# Autodesk Inventor assembly: ring_assembly
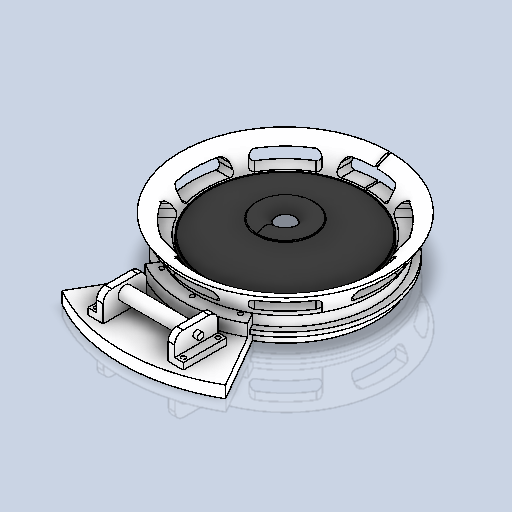
[picture p0: Inventor's stored thumbnail of the model, 512x512]
Saved by Autodesk Inventor 2026.1 (Build 301233000, 233)
## iProperties
Created: 2025-08-31
Part Number: ring_assembly
Document SubType Name: Assembly
Designer: baseb
Author: baseb
## Documents named in this file (7)
- C:\Users\baseb\Desktop\LANL-Glovebox-Closure-Mechanism\ring_assembly.iam
- C:\Users\baseb\Desktop\LANL-Glovebox-Closure-Mechanism\Glove_ring.ipt
- C:\Users\baseb\Desktop\LANL-Glovebox-Closure-Mechanism\shelf_attachment.ipt
- C:\Users\baseb\Desktop\LANL-Glovebox-Closure-Mechanism\drum_holder.ipt
- C:\Users\baseb\Desktop\LANL-Glovebox-Closure-Mechanism\drum.ipt
- C:\Users\baseb\Desktop\LANL-Glovebox-Closure-Mechanism\rubber_sleeve.ipt
- C:\Users\baseb\Desktop\LANL-Glovebox-Closure-Mechanism\rubber_sleeve_open.ipt
## Components (7 placed, 6 different names)
1. Glove_ring:1 — Mate:1, Flush:1, Mate:10, Mate:11, Mate:12, Mate:13
2. shelf_attachment:1 — Mate:1, Flush:1, Mate:2, Mate:3, Mate:4, Mate:5, Mate:6, Mate:7
3. drum_holder:1 — Mate:5, Mate:6, Mate:7
4. drum_holder:2 — Mate:2, Mate:3, Mate:4, Mate:8, Mate:9
5. drum:1 — Mate:8, Mate:9
6. rubber_sleeve:1 — Mate:10, Mate:11
7. rubber_sleeve_open:1 — Mate:12, Mate:13
## Relationships (14: Mate 13, Flush 1)
- Mate:1: Glove_ring:1 ↔ shelf_attachment:1
- Flush:1: Glove_ring:1 ↔ shelf_attachment:1
- Mate:2: shelf_attachment:1 ↔ drum_holder:2
- Mate:3: shelf_attachment:1 ↔ drum_holder:2
- Mate:4: shelf_attachment:1 ↔ drum_holder:2
- Mate:5: shelf_attachment:1 ↔ drum_holder:1
- Mate:6: shelf_attachment:1 ↔ drum_holder:1
- Mate:7: shelf_attachment:1 ↔ drum_holder:1
- Mate:8: drum_holder:2 ↔ drum:1
- Mate:9: drum_holder:2 ↔ drum:1
- Mate:10: Glove_ring:1 ↔ rubber_sleeve:1
- Mate:11: Glove_ring:1 ↔ rubber_sleeve:1
- Mate:12: Glove_ring:1 ↔ rubber_sleeve_open:1
- Mate:13: Glove_ring:1 ↔ rubber_sleeve_open:1
